# Autodesk Inventor assembly: PCB_VUC
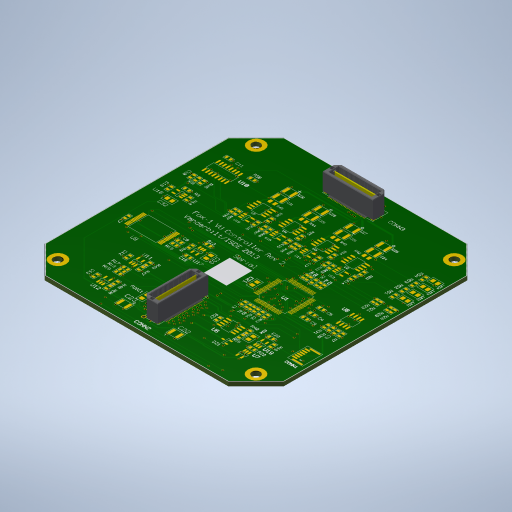
[picture p0: Inventor's stored thumbnail of the model, 512x512]
Saved by Autodesk Inventor 2023 (Build 270158000, 158)
## iProperties
Created: 2011-10-12
Part Number: PCB_VUC
Document SubType Name: Assembly
Designer: Robert Davis
Description: EXPERIMENT #1 PCB
Mass: 35.2633 g
Surface Area: 354.09 cm^2
Volume: 16.1818 cm^3
Density: 2.17919 g/cm^3
Author: Robert Davis
## Documents named in this file (5)
- E:\Dropbox\AMSAT\CAD_backup_frequent_files_20200629\PCB_VUC.iam
- E:\Dropbox\AMSAT\CAD_backup_frequent_files_20200629\Samtec_QSH-030-01-L-D-A.ipt
- E:\Dropbox\AMSAT\CAD_backup_frequent_files_20200629\Samtec_QTH-030-02-L-D-A.ipt
- E:\Dropbox\AMSAT\CAD_backup_frequent_files_20200629\Exp1_extramass.ipt
- E:\Dropbox\AMSAT\CAD_backup_frequent_files_20200629\PCB_VUC.ipt
## Components (5 placed, 4 different names)
1. PCB_VUC:1 — Mate:3, Mate:4, Angle:3, Mate:1, Mate:2, Angle:4, Mate:5
2. Samtec_QTH-030-02-L-D-A:1 — Mate:1, Mate:2, Angle:4
3. Samtec_QSH-030-01-L-D-A:1 — Mate:3, Mate:4, Angle:3
4. Samtec_QTH-030-02-L-D-A:2 — Mate:5, Mate:6
5. Exp1_extramass:1 — Flush:2, Flush:3, Flush:4
## Relationships (12: Mate 6, Flush 4, Angle 2)
- Mate:3: PCB_VUC:1 ↔ Samtec_QSH-030-01-L-D-A:1
- Mate:4: PCB_VUC:1 ↔ Samtec_QSH-030-01-L-D-A:1
- Angle:3 (180 deg): PCB_VUC:1 ↔ Samtec_QSH-030-01-L-D-A:1
- Mate:1: PCB_VUC:1 ↔ Samtec_QTH-030-02-L-D-A:1
- Mate:2: PCB_VUC:1 ↔ Samtec_QTH-030-02-L-D-A:1
- Angle:4 (180 deg): PCB_VUC:1 ↔ Samtec_QTH-030-02-L-D-A:1
- Mate:5: PCB_VUC:1 ↔ Samtec_QTH-030-02-L-D-A:2
- [Flush]: Samtec_QTH-030-02-L-D-A:2
- Mate:6 (39.5 mm): Samtec_QTH-030-02-L-D-A:2
- Flush:2: Exp1_extramass:1
- Flush:3: Exp1_extramass:1
- Flush:4: Exp1_extramass:1
